# Autodesk Inventor assembly: 2 Falcon Reverse Mount V2 (WCP-0496)
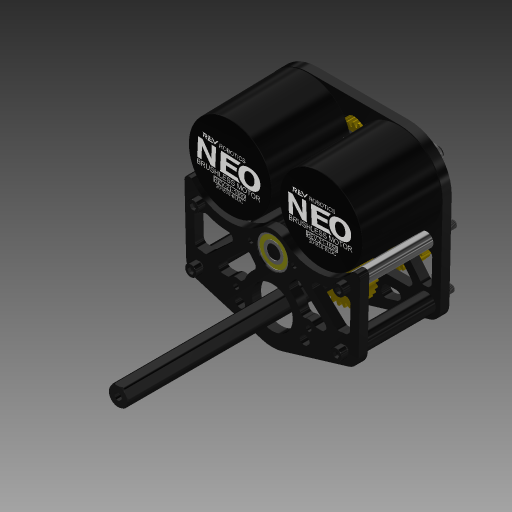
[picture p0: Inventor's stored thumbnail of the model, 512x512]
Saved by Autodesk Inventor 2023 (Build 270158000, 158)
## iProperties
Created: 2023-03-18
Part Number: 2 Falcon Reverse Mount V2 (WCP-0496)
Document SubType Name: Assembly
Designer: Max Boord
Mass: 1460.1 g
Surface Area: 1506.32 cm^2
Volume: 489.505 cm^3
Density: 2.98282 g/cm^3
Author: Max Boord
## Documents named in this file (28)
- E:\Collaborative Robots\Collaborative Part Library\Drivetrains\COTS WCD Gearboxes\2 Falcon Reverse Mount V2 (WCP-0496)\2 Falcon Reverse Mount V2 (WCP-0496).iam
- E:\Collaborative Robots\Collaborative Part Library\Drivetrains\COTS WCD Gearboxes\2 Falcon Reverse Mount V2 (WCP-0496)\Gearbox Output Shaft (WCP-0832).ipt
- E:\Collaborative Robots\Collaborative Part Library\Drivetrains\COTS WCD Gearboxes\2 Falcon Reverse Mount V2 (WCP-0496)\WCP-0496-001 Rev2.ipt
- E:\Collaborative Robots\Collaborative Part Library\Drivetrains\COTS WCD Gearboxes\2 Falcon Reverse Mount V2 (WCP-0496)\WCP-0496-002 Rev2.ipt
- E:\Collaborative Robots\Collaborative Part Library\Drivetrains\COTS WCD Gearboxes\2 Falcon Reverse Mount V2 (WCP-0496)\WCP-0496-003 Rev2.ipt
- E:\Collaborative Robots\Collaborative Part Library\Drivetrains\COTS WCD Gearboxes\2 Falcon Reverse Mount V2 (WCP-0496)\WCP-0566 Rev1.ipt
- E:\Collaborative Robots\Collaborative Part Library\Power Transfer\Bearings and Bushings\Bearings\FR8 (Thunderhex).ipt
- E:\Collaborative Robots\Collaborative Part Library\Power Transfer\Bearings and Bushings\Bearings.ipt
- E:\Collaborative Robots\Collaborative Part Library\Power Transfer\Bearings and Bushings\Bearings\FR6.ipt
- E:\Collaborative Robots\Collaborative Part Library\Power Transfer\Bearings and Bushings\Bearings\FR8.ipt
- E:\Collaborative Robots\Collaborative Part Library\Motors\FRC\NEO.ipt
- E:\Collaborative Robots\Collaborative Part Library\Motors\FRC\Motor Pinions.ipt
- E:\Collaborative Robots\Collaborative Part Library\Hardware\Spacers\REV CIM Motor Shaft Spacer (REV-21-2078).ipt
- E:\Collaborative Robots\Collaborative Part Library\Hardware\Fasteners\Machine Screws\10-32 UNFx0.25 Button Head Cap Screw.ipt
- E:\Collaborative Robots\Collaborative Part Library\Hardware\Fasteners\Machine Screws.ipt
- E:\Collaborative Robots\Collaborative Part Library\Power Transfer\Gears (Hex)\Spur Gear2\20dp 62T VexPro 500 Hex Aluminum Gear (Pocketed).ipt
- E:\Collaborative Robots\Collaborative Part Library\Power Transfer\Gears (Hex)\VexPro Spur Gears.ipt
- E:\Collaborative Robots\Collaborative Part Library\Hardware\Spacers\Spacers & Standoffs\WCP Aluminum Standoff (No. 10 x 2Lg x 0.375OD).ipt
- E:\Collaborative Robots\Collaborative Part Library\Hardware\Spacers\Spacers & Standoffs.ipt
- E:\Collaborative Robots\Collaborative Part Library\Power Transfer\Gears (Hex)\Spur Gear2\20dp 22T VexPro 500 Hex Steel Gear.ipt
- E:\Collaborative Robots\Collaborative Part Library\Power Transfer\Gears (Hex)\Spur Gear2\20dp 30T VexPro 500 Hex Aluminum Gear.ipt
- E:\Collaborative Robots\Collaborative Part Library\Shaft Retention\Snaprings\Snapring for 0.5in Shaft (0.461in).ipt
- E:\Collaborative Robots\Collaborative Part Library\Shaft Retention\Snaprings.ipt
- E:\Collaborative Robots\Collaborative Part Library\Hardware\Spacers\Hex Spacers.ipt
- E:\Collaborative Robots\Collaborative Part Library\Hardware\Nuts and Threaded Blocks\Nuts\10-32 Pan Head Nylon locknut.ipt
- E:\Collaborative Robots\Collaborative Part Library\Hardware\Nuts and Threaded Blocks\Nuts.ipt
- E:\Collaborative Robots\Collaborative Part Library\Hardware\Fasteners\Machine Screws\10-32 UNFx3 Socket Head Cap Screw.ipt
- E:\Collaborative Robots\Collaborative Part Library\Hardware\Fasteners\Machine Screws\10-32 UNFx0.5 Button Head Cap Screw.ipt
## Components (43 placed, 21 different names)
1. Gearbox Output Shaft (WCP-0832):1 — Mate:3, Insert:9, Insert:25
2. WCP-0496-001 Rev2:1 — Mate:2, Mate:3, Mate:4, Insert:2, Insert:3, Insert:5, Insert:8, Insert:10, Insert:11, Insert:21, Insert:22, Insert:26, Insert:27, Insert:31, Insert:32, Insert:33, Insert:34, Insert:39, Insert:40, Insert:41, Insert:42, Insert:43, Insert:44
3. WCP-0496-002 Rev2:1 — Mate:1, Flush:1, Mate:2, Insert:1, Flush:2, Insert:4, Insert:6, Insert:28, Insert:29, Insert:35, Insert:36, Insert:37, Insert:38
4. WCP-0496-003 Rev2:1 — Mate:4, Insert:7, Insert:20, Insert:24
5. WCP-0566 Rev1:1 — Insert:3, Insert:4
6. WCP-0566 Rev1:2 — Insert:1, Insert:2
7. FR8 (Thunderhex):1 — Insert:5, Insert:23, Insert:30
8. FR6:2 — Insert:6, Insert:7
9. FR8:3 — Insert:8, Insert:9, Mate:5
10. NEO:1 — Insert:11, Insert:15, Insert:18, Insert:39
11. NEO:2 — Insert:10, Insert:13, Insert:19, Insert:40
12. Motor Pinions:1 — Insert:12, Insert:17
13. REV CIM Motor Shaft Spacer (REV-21-2078):1 — Insert:12, Insert:13
14. Motor Pinions:2 — Insert:16
15. REV CIM Motor Shaft Spacer (REV-21-2078):2 — Insert:15
16. REV CIM Motor Shaft Spacer (REV-21-2078):3 — Insert:16
17. REV CIM Motor Shaft Spacer (REV-21-2078):4 — Insert:17
18. 10-32 UNFx0.25 Button Head Cap Screw:1 — Insert:18
19. 10-32 UNFx0.25 Button Head Cap Screw:2 — Insert:19
20. 20dp 62T VexPro 500 Hex Aluminum Gear (Pocketed):1 — Insert:20
21. WCP Aluminum Standoff (No. 10 x 2Lg x 0.375OD):1 — Insert:22
22. WCP Aluminum Standoff (No. 10 x 2Lg x 0.375OD):2 — Insert:21
23. 20dp 22T VexPro 500 Hex Steel Gear:2 — Insert:23, Flush:4
24. 20dp 30T VexPro 500 Hex Aluminum Gear:3 — Flush:4, Mate:5
25. Snapring for 0.5in Shaft (0.461in):1 — Insert:24
26. Snapring for 0.5in Shaft (0.461in):2 — Insert:25
27. 10-32 UNFx0.25 Button Head Cap Screw:3 — Insert:26
28. 10-32 UNFx0.25 Button Head Cap Screw:4 — Insert:27
29. 10-32 UNFx0.25 Button Head Cap Screw:5 — Insert:29
30. 10-32 UNFx0.25 Button Head Cap Screw:6 — Insert:28
31. Hex Spacers:1 — Insert:30
32. 10-32 Pan Head Nylon locknut:1 — Insert:32
33. 10-32 Pan Head Nylon locknut:2 — Insert:33
34. 10-32 Pan Head Nylon locknut:3 — Insert:34
35. 10-32 Pan Head Nylon locknut:4 — Insert:31
36. 10-32 UNFx3 Socket Head Cap Screw:7 — Insert:35
37. 10-32 UNFx3 Socket Head Cap Screw:8 — Insert:36
38. 10-32 UNFx3 Socket Head Cap Screw:9 — Insert:37
39. 10-32 UNFx3 Socket Head Cap Screw:10 — Insert:38
40. 10-32 UNFx0.5 Button Head Cap Screw:11 — Insert:41
41. 10-32 UNFx0.5 Button Head Cap Screw:12 — Insert:42
42. 10-32 UNFx0.5 Button Head Cap Screw:13 — Insert:43
43. 10-32 UNFx0.5 Button Head Cap Screw:14 — Insert:44
## Relationships (52: Insert 44, Mate 5, Flush 3)
- Mate:1: WCP-0496-002 Rev2:1
- Flush:1: WCP-0496-002 Rev2:1
- Mate:2: WCP-0496-001 Rev2:1 ↔ WCP-0496-002 Rev2:1
- Mate:3: Gearbox Output Shaft (WCP-0832):1 ↔ WCP-0496-001 Rev2:1
- Mate:4: WCP-0496-001 Rev2:1 ↔ WCP-0496-003 Rev2:1
- Insert:1: WCP-0496-002 Rev2:1 ↔ WCP-0566 Rev1:2
- Insert:2: WCP-0496-001 Rev2:1 ↔ WCP-0566 Rev1:2
- Flush:2: WCP-0496-002 Rev2:1
- Insert:3: WCP-0496-001 Rev2:1 ↔ WCP-0566 Rev1:1
- Insert:4: WCP-0496-002 Rev2:1 ↔ WCP-0566 Rev1:1
- Insert:5: WCP-0496-001 Rev2:1 ↔ FR8 (Thunderhex):1
- Insert:6: WCP-0496-002 Rev2:1 ↔ FR6:2
- Insert:7: WCP-0496-003 Rev2:1 ↔ FR6:2
- Insert:8: WCP-0496-001 Rev2:1 ↔ FR8:3
- Insert:9: Gearbox Output Shaft (WCP-0832):1 ↔ FR8:3
- Insert:10: WCP-0496-001 Rev2:1 ↔ NEO:2
- Insert:11: WCP-0496-001 Rev2:1 ↔ NEO:1
- Insert:12: Motor Pinions:1 ↔ REV CIM Motor Shaft Spacer (REV-21-2078):1
- Insert:13: NEO:2 ↔ REV CIM Motor Shaft Spacer (REV-21-2078):1
- [Insert]: Motor Pinions:2 ↔ REV CIM Motor Shaft Spacer (REV-21-2078):2
- Insert:15: NEO:1 ↔ REV CIM Motor Shaft Spacer (REV-21-2078):2
- Insert:16: Motor Pinions:2 ↔ REV CIM Motor Shaft Spacer (REV-21-2078):3
- Insert:17: Motor Pinions:1 ↔ REV CIM Motor Shaft Spacer (REV-21-2078):4
- Insert:18: NEO:1 ↔ 10-32 UNFx0.25 Button Head Cap Screw:1
- Insert:19: NEO:2 ↔ 10-32 UNFx0.25 Button Head Cap Screw:2
- Insert:20: WCP-0496-003 Rev2:1 ↔ 20dp 62T VexPro 500 Hex Aluminum Gear (Pocketed):1
- Insert:21: WCP-0496-001 Rev2:1 ↔ WCP Aluminum Standoff (No. 10 x 2Lg x 0.375OD):2
- Insert:22: WCP-0496-001 Rev2:1 ↔ WCP Aluminum Standoff (No. 10 x 2Lg x 0.375OD):1
- Insert:23: FR8 (Thunderhex):1 ↔ 20dp 22T VexPro 500 Hex Steel Gear:2
- Flush:4: 20dp 22T VexPro 500 Hex Steel Gear:2 ↔ 20dp 30T VexPro 500 Hex Aluminum Gear:3
- Mate:5: FR8:3 ↔ 20dp 30T VexPro 500 Hex Aluminum Gear:3
- Insert:24: WCP-0496-003 Rev2:1 ↔ Snapring for 0.5in Shaft (0.461in):1
- Insert:25: Gearbox Output Shaft (WCP-0832):1 ↔ Snapring for 0.5in Shaft (0.461in):2
- Insert:26 (1.5875 mm): WCP-0496-001 Rev2:1 ↔ 10-32 UNFx0.25 Button Head Cap Screw:3
- Insert:27 (1.5875 mm): WCP-0496-001 Rev2:1 ↔ 10-32 UNFx0.25 Button Head Cap Screw:4
- Insert:28 (1.5875 mm): WCP-0496-002 Rev2:1 ↔ 10-32 UNFx0.25 Button Head Cap Screw:6
- Insert:29 (1.5875 mm): WCP-0496-002 Rev2:1 ↔ 10-32 UNFx0.25 Button Head Cap Screw:5
- Insert:30: FR8 (Thunderhex):1 ↔ Hex Spacers:1
- Insert:31: WCP-0496-001 Rev2:1 ↔ 10-32 Pan Head Nylon locknut:4
- Insert:32: WCP-0496-001 Rev2:1 ↔ 10-32 Pan Head Nylon locknut:1
- Insert:33: WCP-0496-001 Rev2:1 ↔ 10-32 Pan Head Nylon locknut:2
- Insert:34: WCP-0496-001 Rev2:1 ↔ 10-32 Pan Head Nylon locknut:3
- Insert:35: WCP-0496-002 Rev2:1 ↔ 10-32 UNFx3 Socket Head Cap Screw:7
- Insert:36: WCP-0496-002 Rev2:1 ↔ 10-32 UNFx3 Socket Head Cap Screw:8
- Insert:37 (1.5875 mm): WCP-0496-002 Rev2:1 ↔ 10-32 UNFx3 Socket Head Cap Screw:9
- Insert:38 (1.5875 mm): WCP-0496-002 Rev2:1 ↔ 10-32 UNFx3 Socket Head Cap Screw:10
- Insert:39: WCP-0496-001 Rev2:1 ↔ NEO:1
- Insert:40: WCP-0496-001 Rev2:1 ↔ NEO:2
- Insert:41: WCP-0496-001 Rev2:1 ↔ 10-32 UNFx0.5 Button Head Cap Screw:11
- Insert:42: WCP-0496-001 Rev2:1 ↔ 10-32 UNFx0.5 Button Head Cap Screw:12
- Insert:43: WCP-0496-001 Rev2:1 ↔ 10-32 UNFx0.5 Button Head Cap Screw:13
- Insert:44: WCP-0496-001 Rev2:1 ↔ 10-32 UNFx0.5 Button Head Cap Screw:14
## Named parameters: d20_d18 = 0 mm
